# Autodesk Inventor assembly: Assembly1
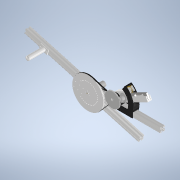
[picture p0: Inventor's stored thumbnail of the model, 180x180]
Saved by Autodesk Inventor 2022.3 (Build 263350000, 350)
## iProperties
Created: 2022-01-28
Part Number: Assembly1
Document SubType Name: Assembly
Designer: Martijn
Author: Martijn
## Documents named in this file (23)
- D:\phd\git\1dofsetup\Assembly1.iam
- D:\phd\git\1dofsetup\30x30x50.ipt
- D:\phd\git\1dofsetup\bearing_mount.ipt
- D:\phd\git\1dofsetup\force_measurement_thingy.ipt
- D:\phd\git\1dofsetup\NEMA 17.ipt
- D:\phd\git\1dofsetup\pololu-universal-aluminum-mounting-hub-for-5mm-shaft-m3-holes.ipt
- D:\phd\git\1dofsetup\space_plate.ipt
- D:\phd\git\1dofsetup\pololu-universal-aluminum-mounting-hub-for-8mm-shaft-m3-holes.ipt
- D:\phd\git\1dofsetup\SKF_608-2ZZ.ipt
- D:\phd\git\1dofsetup\just_pulley.ipt
- D:\phd\git\1dofsetup\force_measurement_plate.ipt
- D:\phd\git\1dofsetup\load_cell.ipt
- D:\phd\git\1dofsetup\fixation_circle.ipt
- D:\phd\git\1dofsetup\fixation_plate2.ipt
- D:\phd\git\1dofsetup\8mm_to 6.35mm_kaplin.ipt
- D:\phd\git\1dofsetup\axis1.ipt
- D:\phd\git\1dofsetup\Lock Collar 8mm.ipt
- D:\phd\git\1dofsetup\belt.ipt
- D:\phd\git\1dofsetup\handle.ipt
- D:\phd\git\1dofsetup\bearing_mount3.ipt
- D:\phd\git\1dofsetup\axis2.ipt
- D:\phd\git\1dofsetup\load_cell_mounting_block2.ipt
- D:\phd\git\1dofsetup\gear1.ipt
## Components (26 placed, 22 different names)
1. 30x30x50:1 — Mate:96, Flush:34, Mate:106, Flush:35, Flush:36, Mate:118, Flush:38, Mate:131, Flush:44, Mate:132, Mate:133
2. 30x30x50:2 — Mate:29, Flush:10, Mate:107, Mate:108, Flush:37, Flush:39, Mate:120, Flush:40
3. force_measurement_thingy:1 — Mate:99, Mate:100, Mate:101, Mate:102, Mate:103, Mate:104, Mate:135, Angle:1
4. NEMA 17:1 — Mate:6, Mate:102, Mate:103, Mate:104, Mate:143, Mate:146
5. pololu-universal-aluminum-mounting-hub-for-5mm-shaft-m3-holes:1 — Mate:6, Mate:143, Mate:144, Mate:145
6. space_plate:1 — Flush:39, Mate:120, Flush:40, Mate:124, Flush:41, Flush:42
7. pololu-universal-aluminum-mounting-hub-for-8mm-shaft-m3-holes:1 — Mate:115, Mate:116, Mate:117, Mate:123, Flush:43
8. SKF_608-2ZZ:2 — Mate:136
9. just_pulley:1 — Mate:106, Flush:35, Mate:109, Mate:110, Mate:111, Mate:113, Mate:115, Mate:116, Mate:117, Flush:36, Mate:127, Mate:128, Mate:130
10. SKF_608-2ZZ:4 — Mate:110, Mate:127
11. force_measurement_plate:2 — Mate:29, Flush:10, Mate:78, Mate:100, Mate:134, Mate:137, Mate:138
12. load_cell:1 — Mate:101, Mate:135, Angle:1
13. fixation_circle:1 — Mate:144, Mate:145, Mate:146, Flush:45
14. fixation_plate2:1 — Mate:118, Flush:38, Mate:122, Mate:125, Mate:126, Mate:133
15. 8mm_to 6.35mm_kaplin:1 — Mate:122, Mate:129
16. bearing_mount:1 — Mate:107, Mate:108, Mate:109, Mate:111, Flush:37
17. axis1:1 — Mate:77, Flush:30, Mate:99, Mate:136, Mate:141, Mate:147
18. Lock Collar 8mm:2 — Mate:77, Mate:78, Flush:30, Mate:134
19. belt:1 — Mate:113, Mate:130, Mate:141
20. handle:1 — Mate:96, Flush:34, Mate:123
21. bearing_mount3:1 — Mate:124, Flush:41, Flush:42, Mate:129
22. SKF_608-2ZZ:5 — Mate:125, Mate:126
23. axis2:1 — Mate:128, Flush:43, Mate:140
24. 30x30x50:3 — Mate:131, Flush:44, Mate:132
25. load_cell_mounting_block2:1 — Mate:137, Mate:138
26. gear1:1 — Mate:147, Flush:45
## Relationships (62: Mate 47, Flush 14, Angle 1)
- Mate:6 (2 mm): NEMA 17:1 ↔ pololu-universal-aluminum-mounting-hub-for-5mm-shaft-m3-holes:1
- Mate:29: 30x30x50:2 ↔ force_measurement_plate:2
- Flush:10: 30x30x50:2 ↔ force_measurement_plate:2
- Mate:77: axis1:1 ↔ Lock Collar 8mm:2
- Mate:78: force_measurement_plate:2 ↔ Lock Collar 8mm:2
- Flush:30 (0.5 mm): axis1:1 ↔ Lock Collar 8mm:2
- Mate:96: 30x30x50:1 ↔ handle:1
- Flush:34: 30x30x50:1 ↔ handle:1
- Mate:99: force_measurement_thingy:1 ↔ axis1:1
- Mate:100 (0.5 mm): force_measurement_thingy:1 ↔ force_measurement_plate:2
- Mate:101: force_measurement_thingy:1 ↔ load_cell:1
- Mate:102: force_measurement_thingy:1 ↔ NEMA 17:1
- Mate:103: force_measurement_thingy:1 ↔ NEMA 17:1
- Mate:104: force_measurement_thingy:1 ↔ NEMA 17:1
- Mate:106: 30x30x50:1 ↔ just_pulley:1
- Flush:35: 30x30x50:1 ↔ just_pulley:1
- Mate:107: 30x30x50:2 ↔ bearing_mount:1
- Mate:108 (-50 mm): 30x30x50:2 ↔ bearing_mount:1
- Mate:109: just_pulley:1 ↔ bearing_mount:1
- Mate:110: just_pulley:1 ↔ SKF_608-2ZZ:4
- Mate:111: just_pulley:1 ↔ bearing_mount:1
- Mate:113: just_pulley:1 ↔ belt:1
- Mate:115: pololu-universal-aluminum-mounting-hub-for-8mm-shaft-m3-holes:1 ↔ just_pulley:1
- Mate:116: pololu-universal-aluminum-mounting-hub-for-8mm-shaft-m3-holes:1 ↔ just_pulley:1
- Mate:117: pololu-universal-aluminum-mounting-hub-for-8mm-shaft-m3-holes:1 ↔ just_pulley:1
- Flush:36: 30x30x50:1 ↔ just_pulley:1
- Flush:37: 30x30x50:2 ↔ bearing_mount:1
- Mate:118: 30x30x50:1 ↔ fixation_plate2:1
- Flush:38: 30x30x50:1 ↔ fixation_plate2:1
- Flush:39: 30x30x50:2 ↔ space_plate:1
- Mate:120: 30x30x50:2 ↔ space_plate:1
- Flush:40: 30x30x50:2 ↔ space_plate:1
- Mate:122: fixation_plate2:1 ↔ 8mm_to 6.35mm_kaplin:1
- Mate:123 (300 mm): pololu-universal-aluminum-mounting-hub-for-8mm-shaft-m3-holes:1 ↔ handle:1
- Mate:124: space_plate:1 ↔ bearing_mount3:1
- Flush:41: space_plate:1 ↔ bearing_mount3:1
- Flush:42: space_plate:1 ↔ bearing_mount3:1
- Mate:125: fixation_plate2:1 ↔ SKF_608-2ZZ:5
- Mate:126: fixation_plate2:1 ↔ SKF_608-2ZZ:5
- Mate:127 (0.5 mm): just_pulley:1 ↔ SKF_608-2ZZ:4
- Mate:128: just_pulley:1 ↔ axis2:1
- Flush:43: pololu-universal-aluminum-mounting-hub-for-8mm-shaft-m3-holes:1 ↔ axis2:1
- Mate:129 (5 mm): 8mm_to 6.35mm_kaplin:1 ↔ bearing_mount3:1
- Mate:130 (0.5 mm): just_pulley:1 ↔ belt:1
- Mate:131: 30x30x50:1 ↔ 30x30x50:3
- Flush:44: 30x30x50:1 ↔ 30x30x50:3
- Mate:132 (-60 mm): 30x30x50:1 ↔ 30x30x50:3
- Mate:133 (-60 mm): 30x30x50:1 ↔ fixation_plate2:1
- Mate:134: force_measurement_plate:2 ↔ Lock Collar 8mm:2
- Mate:135: force_measurement_thingy:1 ↔ load_cell:1
- Mate:136: SKF_608-2ZZ:2 ↔ axis1:1
- Angle:1 (-180 deg): force_measurement_thingy:1 ↔ load_cell:1
- Mate:137: force_measurement_plate:2 ↔ load_cell_mounting_block2:1
- Mate:138: force_measurement_plate:2 ↔ load_cell_mounting_block2:1
- Mate:140: axis2:1
- Mate:141: axis1:1 ↔ belt:1
- Mate:143: NEMA 17:1 ↔ pololu-universal-aluminum-mounting-hub-for-5mm-shaft-m3-holes:1
- Mate:144: pololu-universal-aluminum-mounting-hub-for-5mm-shaft-m3-holes:1 ↔ fixation_circle:1
- Mate:145: pololu-universal-aluminum-mounting-hub-for-5mm-shaft-m3-holes:1 ↔ fixation_circle:1
- Mate:146: NEMA 17:1 ↔ fixation_circle:1
- Mate:147: axis1:1 ↔ gear1:1
- Flush:45 (0.5 mm): fixation_circle:1 ↔ gear1:1
